# Autodesk Inventor assembly: SpringContact_5mm
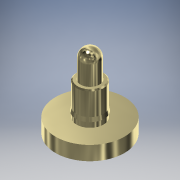
[picture p0: Inventor's stored thumbnail of the model, 180x180]
Saved by Autodesk Inventor 2018 (Build 220112000, 112)
## iProperties
Created: 2018-11-03
Part Number: SpringContact_5mm
Document SubType Name: Assembly
Designer: Bradley
Author: Bradley
## Documents named in this file (3)
- C:\Users\Bradley\Documents\GitHub\Resources\ComponentModels\Electronics\SpringContact_5mm.iam
- C:\Users\Bradley\Documents\GitHub\Resources\ComponentModels\Electronics\Components\SpringContact_5mm\Base.ipt
- C:\Users\Bradley\Documents\GitHub\Resources\ComponentModels\Electronics\Components\SpringContact_5mm\Plunger.ipt
## Components (2 placed, 2 different names)
1. Base:1 — Insert:1
2. Plunger:1 — Insert:1
## Relationships (1: Insert 1)
- Insert:1 (-0.9271 mm): Base:1 ↔ Plunger:1
